# Autodesk Inventor assembly: tmp
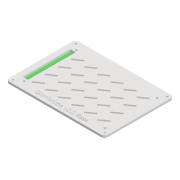
[picture p0: Inventor's stored thumbnail of the model, 180x180]
Saved by Autodesk Inventor 2022 (Build 260153000, 153)
## iProperties
Created: 2023-02-22
Part Number: tmp
Document SubType Name: Assembly
Designer: diederichbenedict
Author: diederichbenedict
## Documents named in this file (3)
- C:\Users\diederichbenedict\Dropbox\Dokumente\Promotion\PROJECTS\Omniscope\INVENTOR\tmp.iam
- C:\Users\diederichbenedict\Dropbox\Dokumente\Promotion\PROJECTS\Omniscope\KiCAD\omniscope\omniscope1.ipt
- C:\Users\diederichbenedict\Dropbox\Dokumente\Promotion\PROJECTS\Omniscope\INVENTOR\Omniscope_2.0_Base.ipt
## Components (2 placed, 2 different names)
1. omniscope1:1 — Einfügen:1, Winkel:1
2. Omniscope_2.0_Base:1 — Einfügen:1, Winkel:1
## Relationships (2: Insert 1, Angle 1)
- Einfügen:1 [Insert]: omniscope1:1 ↔ Omniscope_2.0_Base:1
- Winkel:1 [Angle] (180 deg): omniscope1:1 ↔ Omniscope_2.0_Base:1
